# Autodesk Inventor assembly: Selection_Ramp 1 2 Lanes
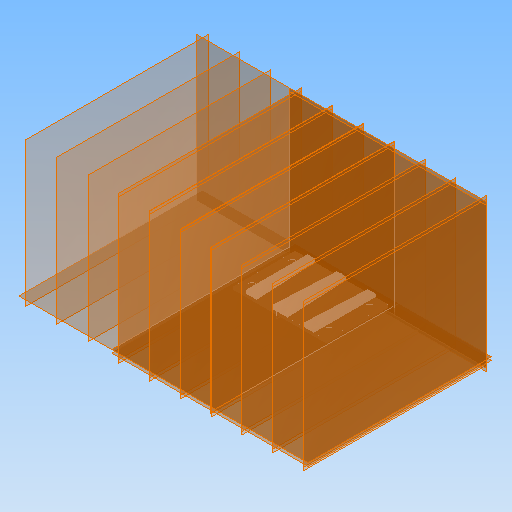
[picture p0: Inventor's stored thumbnail of the model, 512x512]
Saved by Autodesk Inventor 2018.1 (Build 221171000, 171)
## iProperties
Created: 2019-02-07
Part Number: Selection_Ramp 1 2 Lanes
Document SubType Name: Assembly
Designer: James
Author: James
## Documents named in this file (9)
- C:\Users\admin\Desktop\Ball-Machine\Selection Sort\Selection - 2 Lanes\Selection_Ramp 1 2 Lanes.iam
- C:\Users\admin\Desktop\Ball-Machine\Selection Sort\Selection_Ramp 1_LHS Piece.ipt
- C:\Users\admin\Desktop\Ball-Machine\Selection Sort\Selection_Ramp 1_Mid piece.ipt
- C:\Users\admin\Desktop\Ball-Machine\Prototype CAD\Selection Sort - 40mm\Nyloc Nut - M4.ipt
- C:\Users\admin\Desktop\Ball-Machine\Selection Sort\Selection_Ramp 1_RHS Piece.ipt
- C:\Users\admin\Desktop\Ball-Machine\Prototype CAD\Selection Sort - 40mm\Socket Csk Screw - (A2) - M4 x  16.ipt
- C:\Users\admin\Desktop\Ball-Machine\Selection Sort\Selection_Angle Bracket 1.ipt
- C:\Users\admin\Desktop\Ball-Machine\Prototype CAD\Selection Sort - 40mm\Socket Csk Screw - (A2) - M4 x  12.ipt
- C:\Users\admin\Desktop\Ball-Machine\Selection Sort\Selection - 2 Lanes\Selection_Ramp 1 2 Lanes.ipt
## Components (26 placed, 8 different names)
1. Selection_Ramp 1 2 Lanes:1 — Flush:1, Flush:2, Flush:3, Mate:1, Mate:2, Mate:3, Flush:4, Flush:5, Mate:4, Flush:6, Flush:7, Mate:5, Mate:6, Mate:7, Flush:8, Flush:9, Mate:14, Mate:15, Mate:18, Mate:19, Mate:20, Mate:21, Mate:22, Flush:10, Mate:23, Mate:24, Mate:25, Mate:26, Tangent:3, Tangent:4, Tangent:5, Tangent:6, Mate:35, Mate:36, Mate:37, Flush:11, Mate:38, Mate:39
2. Selection_Ramp 1_RHS Piece:1 — Mate:7, Flush:8, Flush:9, Mate:40
3. Selection_Ramp 1_LHS Piece:2 — Mate:4, Flush:6, Flush:7, Mate:5, Mate:6, Tangent:1, Tangent:2
4. Nyloc Nut - M4:25 — Mate:27, Mate:30
5. Selection_Angle Bracket 1:1 — Mate:22, Flush:10, Mate:23, Mate:24, Mate:27, Mate:28
6. Socket Csk Screw - (A2) - M4 x  12:2 — Mate:25, Tangent:4, Mate:30
7. Nyloc Nut - M4:26 — Mate:28, Mate:29
8. Socket Csk Screw - (A2) - M4 x  12:1 — Mate:26, Tangent:3, Mate:29
9. Nyloc Nut - M4:27
10. Selection_Angle Bracket 1:2 — Mate:37, Flush:11, Mate:38, Mate:39
11. Socket Csk Screw - (A2) - M4 x  12:3 — Tangent:6, Mate:35
12. Nyloc Nut - M4:28
13. Socket Csk Screw - (A2) - M4 x  12:4 — Tangent:5, Mate:36
14. Selection_Ramp 1_Mid piece:1 — Mate:1, Mate:2, Mate:3, Flush:4, Flush:5
15. Socket Csk Screw - (A2) - M4 x  16:1 — Mate:19, Tangent:2
16. Socket Csk Screw - (A2) - M4 x  16:7 — Mate:21, Tangent:1
17. Nyloc Nut - M4:13 — Mate:15, Mate:20
18. Nyloc Nut - M4:19 — Mate:14, Mate:18
19. Socket Csk Screw - (A2) - M4 x  16:2
20. Socket Csk Screw - (A2) - M4 x  16:8
21. Nyloc Nut - M4:14
22. Nyloc Nut - M4:20
23. Socket Csk Screw - (A2) - M4 x  16:3 — Mate:40
24. Socket Csk Screw - (A2) - M4 x  16:9
25. Nyloc Nut - M4:15
26. Nyloc Nut - M4:21
## Component patterns: (1 elements, first: Selection_Ramp 1_Mid piece:1), (3 elements, first: Socket Csk Screw - (A2) - M4 x  16:1 + Socket Csk Screw - (A2) - M4 x  16:7 + Nyloc Nut - M4:13 + Nyloc Nut - M4:19)
## Relationships (49: Mate 32, Flush 11, Tangent 6)
- Flush:1: Selection_Ramp 1 2 Lanes:1
- Flush:2: Selection_Ramp 1 2 Lanes:1
- Flush:3: Selection_Ramp 1 2 Lanes:1
- Mate:1: Selection_Ramp 1 2 Lanes:1 ↔ Selection_Ramp 1_Mid piece:1
- Mate:2: Selection_Ramp 1 2 Lanes:1 ↔ Selection_Ramp 1_Mid piece:1
- Mate:3: Selection_Ramp 1 2 Lanes:1 ↔ Selection_Ramp 1_Mid piece:1
- Flush:4: Selection_Ramp 1 2 Lanes:1 ↔ Selection_Ramp 1_Mid piece:1
- Flush:5: Selection_Ramp 1 2 Lanes:1 ↔ Selection_Ramp 1_Mid piece:1
- Mate:4: Selection_Ramp 1 2 Lanes:1 ↔ Selection_Ramp 1_LHS Piece:2
- Flush:6: Selection_Ramp 1 2 Lanes:1 ↔ Selection_Ramp 1_LHS Piece:2
- Flush:7: Selection_Ramp 1 2 Lanes:1 ↔ Selection_Ramp 1_LHS Piece:2
- Mate:5: Selection_Ramp 1 2 Lanes:1 ↔ Selection_Ramp 1_LHS Piece:2
- Mate:6: Selection_Ramp 1 2 Lanes:1 ↔ Selection_Ramp 1_LHS Piece:2
- Mate:7: Selection_Ramp 1 2 Lanes:1 ↔ Selection_Ramp 1_RHS Piece:1
- Flush:8: Selection_Ramp 1 2 Lanes:1 ↔ Selection_Ramp 1_RHS Piece:1
- Flush:9: Selection_Ramp 1 2 Lanes:1 ↔ Selection_Ramp 1_RHS Piece:1
- Mate:14: Selection_Ramp 1 2 Lanes:1 ↔ Nyloc Nut - M4:19
- Mate:15: Selection_Ramp 1 2 Lanes:1 ↔ Nyloc Nut - M4:13
- Mate:18: Selection_Ramp 1 2 Lanes:1 ↔ Nyloc Nut - M4:19
- Mate:19: Selection_Ramp 1 2 Lanes:1 ↔ Socket Csk Screw - (A2) - M4 x  16:1
- Mate:20: Selection_Ramp 1 2 Lanes:1 ↔ Nyloc Nut - M4:13
- Mate:21: Selection_Ramp 1 2 Lanes:1 ↔ Socket Csk Screw - (A2) - M4 x  16:7
- Tangent:1: Selection_Ramp 1_LHS Piece:2 ↔ Socket Csk Screw - (A2) - M4 x  16:7
- Tangent:2: Selection_Ramp 1_LHS Piece:2 ↔ Socket Csk Screw - (A2) - M4 x  16:1
- Mate:22: Selection_Ramp 1 2 Lanes:1 ↔ Selection_Angle Bracket 1:1
- Flush:10: Selection_Ramp 1 2 Lanes:1 ↔ Selection_Angle Bracket 1:1
- Mate:23: Selection_Ramp 1 2 Lanes:1 ↔ Selection_Angle Bracket 1:1
- Mate:24: Selection_Ramp 1 2 Lanes:1 ↔ Selection_Angle Bracket 1:1
- Mate:25: Selection_Ramp 1 2 Lanes:1 ↔ Socket Csk Screw - (A2) - M4 x  12:2
- Mate:26: Selection_Ramp 1 2 Lanes:1 ↔ Socket Csk Screw - (A2) - M4 x  12:1
- Mate:27: Nyloc Nut - M4:25 ↔ Selection_Angle Bracket 1:1
- Mate:28: Selection_Angle Bracket 1:1 ↔ Nyloc Nut - M4:26
- Tangent:3: Selection_Ramp 1 2 Lanes:1 ↔ Socket Csk Screw - (A2) - M4 x  12:1
- Tangent:4: Selection_Ramp 1 2 Lanes:1 ↔ Socket Csk Screw - (A2) - M4 x  12:2
- Mate:29: Nyloc Nut - M4:26 ↔ Socket Csk Screw - (A2) - M4 x  12:1
- Mate:30: Nyloc Nut - M4:25 ↔ Socket Csk Screw - (A2) - M4 x  12:2
- [Mate]: Nyloc Nut - M4:27 ↔ Selection_Angle Bracket 1:2
- [Mate]: Selection_Angle Bracket 1:2 ↔ Nyloc Nut - M4:28
- [Mate]: Nyloc Nut - M4:28 ↔ Socket Csk Screw - (A2) - M4 x  12:4
- [Mate]: Nyloc Nut - M4:27 ↔ Socket Csk Screw - (A2) - M4 x  12:3
- Tangent:5: Selection_Ramp 1 2 Lanes:1 ↔ Socket Csk Screw - (A2) - M4 x  12:4
- Tangent:6: Selection_Ramp 1 2 Lanes:1 ↔ Socket Csk Screw - (A2) - M4 x  12:3
- Mate:35: Selection_Ramp 1 2 Lanes:1 ↔ Socket Csk Screw - (A2) - M4 x  12:3
- Mate:36: Selection_Ramp 1 2 Lanes:1 ↔ Socket Csk Screw - (A2) - M4 x  12:4
- Mate:37: Selection_Ramp 1 2 Lanes:1 ↔ Selection_Angle Bracket 1:2
- Flush:11: Selection_Ramp 1 2 Lanes:1 ↔ Selection_Angle Bracket 1:2
- Mate:38: Selection_Ramp 1 2 Lanes:1 ↔ Selection_Angle Bracket 1:2
- Mate:39: Selection_Ramp 1 2 Lanes:1 ↔ Selection_Angle Bracket 1:2
- Mate:40: Selection_Ramp 1_RHS Piece:1 ↔ Socket Csk Screw - (A2) - M4 x  16:3
## Named parameters: d52_d46 = 0 mm, d53_d47 = 0 mm, d54_d50 = 0 mm, d55_d51 = 0 mm
